# Autodesk Inventor assembly: assembly
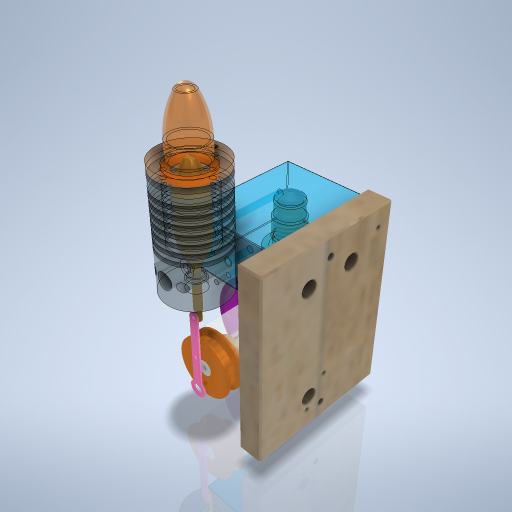
[picture p0: Inventor's stored thumbnail of the model, 512x512]
Saved by Autodesk Inventor 2024.2 (Build 282272000, 272)
## iProperties
Created: 2024-05-01
Part Number: assembly
Document SubType Name: Assembly
Designer: Fabri
Author: Fabri
## Documents named in this file (14)
- C:\Users\Fabri\Documents\Inventor\steam engine\assembly.iam
- C:\Users\Fabri\Documents\Inventor\steam engine\Grundplatte.ipt
- C:\Users\Fabri\Documents\Inventor\steam engine\Steuerblock.ipt
- C:\Users\Fabri\Documents\Inventor\steam engine\Lagerblock.ipt
- C:\Users\Fabri\Documents\Inventor\steam engine\schwingrad.ipt
- C:\Users\Fabri\Documents\Inventor\steam engine\pleuel.ipt
- C:\Users\Fabri\Documents\Inventor\steam engine\arbeitskolben.ipt
- C:\Users\Fabri\Documents\Inventor\steam engine\Arbeitszylinder.ipt
- C:\Users\Fabri\Documents\Inventor\steam engine\poulie.ipt
- C:\Users\Fabri\Documents\Inventor\steam engine\cylinder.ipt
- C:\Users\Fabri\Documents\Inventor\steam engine\steuerkolben.ipt
- C:\Users\Fabri\Documents\Inventor\steam engine\heizrohr.ipt
- C:\Users\Fabri\Documents\Inventor\steam engine\isolatorring.ipt
- C:\Users\Fabri\Documents\Inventor\steam engine\Welle.ipt
## Components (14 placed, 13 different names)
1. Grundplatte:1 — Winkel:1, Einfügen:1, Einfügen:2, Fluchtend:1, Winkel:8
2. Steuerblock:1 — Winkel:1, Einfügen:1, Drehbar:1, Winkel:3, Einfügen:7
3. Lagerblock:1 — Einfügen:2, Winkel:3, Einfügen:3, Einfügen:5
4. schwingrad:1 — Winkel:2, Einfügen:3, Passend:9, Passend:37
5. arbeitskolben:1 — Zylindrisch:1, Einfügen:4
6. Arbeitszylinder:1 — Drehbar:1, Zylindrisch:1
7. pleuel:1 — Einfügen:4, Passend:26
8. poulie:1 — Einfügen:5, Passend:35, Einfügen:8, Winkel:9, Passend:36
9. pleuel:2 — Passend:33, Passend:36
10. cylinder:1 — Einfügen:7, Zylindrisch:2
11. steuerkolben:1 — Zylindrisch:2, Winkel:8, Passend:32
12. heizrohr:1 — Zylindrisch:3, Zylindrisch:4
13. isolatorring:1 — Zylindrisch:3, Zylindrisch:4
14. Welle:2 — Passend:35, Einfügen:8, Winkel:9, Passend:37
## Relationships (31: Mate 13, Insert 7, Angle 5, CylindricalJoint 4, RevoluteJoint 1, Flush 1)
- Winkel:1 [Angle] (0 deg): Grundplatte:1 ↔ Steuerblock:1
- Einfügen:1 [Insert]: Grundplatte:1 ↔ Steuerblock:1
- Winkel:2 [Angle] (720 deg): schwingrad:1
- Drehbar:1 [RevoluteJoint] (-21 mm): Steuerblock:1 ↔ Arbeitszylinder:1
- Zylindrisch:1 [CylindricalJoint]: arbeitskolben:1 ↔ Arbeitszylinder:1
- Einfügen:2 [Insert]: Grundplatte:1 ↔ Lagerblock:1
- Winkel:3 [Angle] (0 deg): Steuerblock:1 ↔ Lagerblock:1
- Einfügen:3 [Insert] (12 mm): Lagerblock:1 ↔ schwingrad:1
- Passend:9 [Mate]: schwingrad:1
- Einfügen:4 [Insert] (0.09 mm): arbeitskolben:1 ↔ pleuel:1
- Einfügen:5 [Insert] (-8 mm): Lagerblock:1 ↔ poulie:1
- Einfügen:7 [Insert]: Steuerblock:1 ↔ cylinder:1
- Zylindrisch:2 [CylindricalJoint]: cylinder:1 ↔ steuerkolben:1
- Passend:18 [Mate]
- Zylindrisch:3 [CylindricalJoint]: heizrohr:1 ↔ isolatorring:1
- Fluchtend:1 [Flush]: Grundplatte:1
- Winkel:8 [Angle] (0 deg): Grundplatte:1 ↔ steuerkolben:1
- Passend:25 [Mate]
- Passend:26 [Mate]: pleuel:1
- Passend:27 [Mate]
- Passend:29 [Mate]
- Passend:31 [Mate]
- Passend:32 [Mate]: steuerkolben:1
- Passend:33 [Mate]: pleuel:2
- Passend:34 [Mate]
- Zylindrisch:4 [CylindricalJoint]: heizrohr:1 ↔ isolatorring:1
- Passend:35 [Mate]: poulie:1 ↔ Welle:2
- Einfügen:8 [Insert] (-58 mm): poulie:1 ↔ Welle:2
- Winkel:9 [Angle] (90 deg): poulie:1 ↔ Welle:2
- Passend:36 [Mate]: poulie:1 ↔ pleuel:2
- Passend:37 [Mate]: schwingrad:1 ↔ Welle:2
